# Autodesk Inventor assembly: GantryDown_MIR1
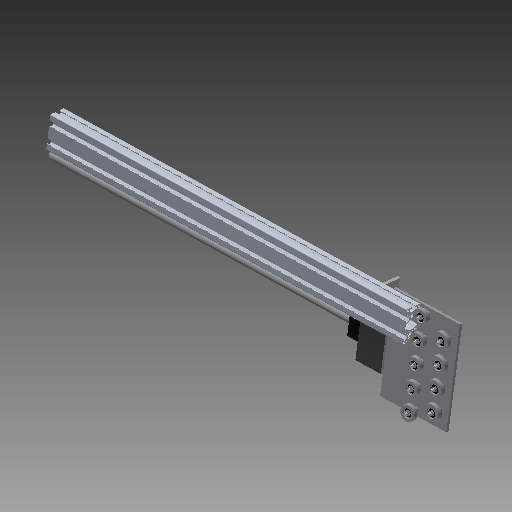
[picture p0: Inventor's stored thumbnail of the model, 512x512]
Saved by Autodesk Inventor 2017 (Build 210142000, 142)
## iProperties
Created: 2016-12-12
Part Number: GantryDown_MIR1
Document SubType Name: Assembly
Designer: umr
Mass: 4376.08 g
Surface Area: 10170.9 cm^2
Volume: 1553.17 cm^3
Density: 2.81752 g/cm^3
Author: umr
## Documents named in this file (9)
- D:\SeniorProject\Models2\Gantry\GantryDown_MIR1.iam
- D:\SeniorProject\Models2\Gantry\ScrewDriver_MIR2.ipt
- D:\SeniorProject\Models2\Gantry\Motor_MIR2.ipt
- D:\SeniorProject\Models2\Gantry\GantryPlate_v3_MIR1.ipt
- D:\SeniorProject\Models2\30x60Sigma_MIR1.ipt
- D:\SeniorProject\Models2\Gantry\M5 Screw with Tee Nut_MIR2.iam
- D:\SeniorProject\Models2\WheelAssembly\OurWheelAssembly_MIR1.iam
- D:\SeniorProject\Models2\WheelAssembly\OurWheelAssemblyBig_MIR1.iam
- D:\SeniorProject\Models2\Gantry\L_Fixer_MIR2.ipt
## Components (21 placed, 8 different names)
1. ScrewDriver_MIR2:1 — Mate:190, Mate:72
2. Motor_MIR2:1 — Mate:190, Mate:72, Flush:3, Mate:197, Flush:2
3. GantryPlate_v3_MIR1:1 — Mate:193, Mate:195, Mate:192, Mate:191, Mate:194, Mate:176, Mate:175, Mate:178, Mate:177, Mate:196
4. 30x60Sigma_MIR1:1 — Mate:193, Mate:171, Mate:157, Mate:170, Mate:158, Mate:165, Mate:159, Mate:166, Mate:160, Mate:186, Mate:184, Mate:181, Mate:183, Mate:182
5. M5 Screw with Tee Nut_MIR2:1 [sub-assembly] — Mate:195, Mate:171, Mate:157
6. M5 Screw with Tee Nut_MIR2:2 [sub-assembly] — Mate:192, Mate:170, Mate:158
7. M5 Screw with Tee Nut_MIR2:3 [sub-assembly] — Mate:191, Mate:165, Mate:159
8. M5 Screw with Tee Nut_MIR2:4 [sub-assembly] — Mate:194, Mate:166, Mate:160
9. M5 Screw with Tee Nut_MIR2:5 [sub-assembly] — Mate:196
10. L_Fixer_MIR2:1 — Flush:3, Mate:197, Flush:2, Mate:186, Mate:187, Mate:185
11. M5 Screw with Tee Nut_MIR2:6 [sub-assembly] — Mate:187, Mate:184, Mate:181
12. M5 Screw with Tee Nut_MIR2:7 [sub-assembly] — Mate:185, Mate:183, Mate:182
13. OurWheelAssembly_MIR1:1 [sub-assembly] — Mate:176, Mate:175
14. OurWheelAssembly_MIR1:2 [sub-assembly]
15. OurWheelAssembly_MIR1:3 [sub-assembly]
16. OurWheelAssembly_MIR1:4 [sub-assembly]
17. OurWheelAssembly_MIR1:5 [sub-assembly]
18. OurWheelAssemblyBig_MIR1:1 [sub-assembly] — Mate:178, Mate:177
19. OurWheelAssemblyBig_MIR1:2 [sub-assembly]
20. OurWheelAssemblyBig_MIR1:3 [sub-assembly]
21. OurWheelAssemblyBig_MIR1:4 [sub-assembly]
## Component patterns: (5 elements, first: OurWheelAssembly_MIR1:1), (4 elements, first: OurWheelAssemblyBig_MIR1:1)
## Relationships (30: Mate 28, Flush 2)
- Mate:190: ScrewDriver_MIR2:1 ↔ Motor_MIR2:1
- Mate:72: ScrewDriver_MIR2:1 ↔ Motor_MIR2:1
- Mate:193: GantryPlate_v3_MIR1:1 ↔ 30x60Sigma_MIR1:1
- Mate:195: GantryPlate_v3_MIR1:1 ↔ M5 Screw with Tee Nut_MIR2:1
- Mate:171 (3 mm): 30x60Sigma_MIR1:1 ↔ M5 Screw with Tee Nut_MIR2:1
- Mate:157: 30x60Sigma_MIR1:1 ↔ M5 Screw with Tee Nut_MIR2:1
- Mate:192: GantryPlate_v3_MIR1:1 ↔ M5 Screw with Tee Nut_MIR2:2
- Mate:170 (3 mm): 30x60Sigma_MIR1:1 ↔ M5 Screw with Tee Nut_MIR2:2
- Mate:158: 30x60Sigma_MIR1:1 ↔ M5 Screw with Tee Nut_MIR2:2
- Mate:191: GantryPlate_v3_MIR1:1 ↔ M5 Screw with Tee Nut_MIR2:3
- Mate:165 (3 mm): 30x60Sigma_MIR1:1 ↔ M5 Screw with Tee Nut_MIR2:3
- Mate:159: 30x60Sigma_MIR1:1 ↔ M5 Screw with Tee Nut_MIR2:3
- Mate:194: GantryPlate_v3_MIR1:1 ↔ M5 Screw with Tee Nut_MIR2:4
- Mate:166 (3 mm): 30x60Sigma_MIR1:1 ↔ M5 Screw with Tee Nut_MIR2:4
- Mate:160: 30x60Sigma_MIR1:1 ↔ M5 Screw with Tee Nut_MIR2:4
- Mate:176: GantryPlate_v3_MIR1:1 ↔ OurWheelAssembly_MIR1:1
- Mate:175: GantryPlate_v3_MIR1:1 ↔ OurWheelAssembly_MIR1:1
- Mate:178: GantryPlate_v3_MIR1:1 ↔ OurWheelAssemblyBig_MIR1:1
- Mate:177: GantryPlate_v3_MIR1:1 ↔ OurWheelAssemblyBig_MIR1:1
- Mate:196: GantryPlate_v3_MIR1:1 ↔ M5 Screw with Tee Nut_MIR2:5
- Flush:3 (10 mm): Motor_MIR2:1 ↔ L_Fixer_MIR2:1
- Mate:197: Motor_MIR2:1 ↔ L_Fixer_MIR2:1
- Flush:2 (10 mm): Motor_MIR2:1 ↔ L_Fixer_MIR2:1
- Mate:186: 30x60Sigma_MIR1:1 ↔ L_Fixer_MIR2:1
- Mate:187: L_Fixer_MIR2:1 ↔ M5 Screw with Tee Nut_MIR2:6
- Mate:184 (3 mm): 30x60Sigma_MIR1:1 ↔ M5 Screw with Tee Nut_MIR2:6
- Mate:181 (3 mm): 30x60Sigma_MIR1:1 ↔ M5 Screw with Tee Nut_MIR2:6
- Mate:185: L_Fixer_MIR2:1 ↔ M5 Screw with Tee Nut_MIR2:7
- Mate:183 (2 mm): 30x60Sigma_MIR1:1 ↔ M5 Screw with Tee Nut_MIR2:7
- Mate:182 (3 mm): 30x60Sigma_MIR1:1 ↔ M5 Screw with Tee Nut_MIR2:7
